# Autodesk Inventor assembly: Funnel Wheel Clamp V4
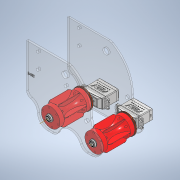
[picture p0: Inventor's stored thumbnail of the model, 180x180]
Saved by Autodesk Inventor 2022 (Build 260153000, 153)
## iProperties
Created: 2022-09-17
Part Number: Funnel Wheel Clamp V4
Document SubType Name: Assembly
Designer: matt
Author: matt
## Documents named in this file (10)
- C:\Users\matt\Documents\Inventor\FTC\2022-23 FTC\Intake\Funnel Wheel Clamp V4.iam
- C:\Users\matt\Documents\Inventor\FTC\2022-23 FTC\FTC Robot Parts\Structural\8mm Bearing with Hex Insert_MIR.iam
- C:\Users\matt\Documents\Inventor\FTC\2022-23 FTC\FTC Robot Parts\Shafts\5mm hex shaft_MIR.ipt
- C:\Users\matt\Documents\Inventor\FTC\2022-23 FTC\FTC Robot Parts\Servos\Servo Horn_MIR.ipt
- C:\Users\matt\Documents\Inventor\FTC\2022-23 FTC\Fasteners\M3 x 8 Button Head.ipt
- C:\Users\matt\Documents\Inventor\FTC\2022-23 FTC\Field\am-4801_Blue Cone.ipt
- C:\Users\matt\Documents\Inventor\FTC\2022-23 FTC\Intake\Intake Sides V5_servo.ipt
- C:\Users\matt\Documents\Inventor\FTC\2022-23 FTC\Motors\REV Smart Servo.ipt
- C:\Users\matt\Documents\Inventor\FTC\2022-23 FTC\Intake\Intake Sides V6ipt.ipt
- C:\Users\matt\Documents\Inventor\FTC\2022-23 FTC\Wheels\Custom Intake Wheel V4.ipt
## Components (19 placed, 9 different names)
1. 8mm Bearing with Hex Insert_MIR:1 [sub-assembly] — Flush:6, Mate:55, Mate:71, Mate:78, Mate:115
2. 8mm Bearing with Hex Insert_MIR:2 [sub-assembly] — Flush:5, Mate:54, Mate:75, Mate:114
3. 5mm hex shaft_MIR:1 — Flush:5, Mate:54, Mate:75, Mate:92
4. 5mm hex shaft_MIR:2 — Flush:6, Mate:55, Mate:71, Mate:72, Mate:93
5. Servo Horn_MIR:1 — Mate:33, Mate:35, Mate:36, Mate:37, Mate:38, Mate:39, Mate:64, Mate:86, Mate:90, Mate:91, Mate:113
6. Servo Horn_MIR:2 — Mate:67, Mate:68, Mate:69, Mate:87, Mate:110
7. M3 x 8 Button Head:1 — Flush:6, Mate:38
8. M3 x 8 Button Head:2 — Flush:6, Flush:7, Mate:39
9. M3 x 8 Button Head:3 — Flush:7, Flush:8, Mate:37
10. M3 x 8 Button Head:4 — Flush:8, Flush:9, Mate:36
11. M3 x 8 Button Head:5 — Flush:9, Flush:10, Mate:35
12. M3 x 8 Button Head:6 — Flush:10, Mate:33, Mate:90
13. Custom Intake Wheel V4:1 — Mate:67, Mate:68, Mate:69, Mate:114
14. Custom Intake Wheel V4:2 — Mate:64, Mate:72, Mate:78, Flush:14, Mate:113
15. am-4801_Blue Cone:1 — Mate:81, Mate:94
16. Intake Sides V5_servo:2 — Mate:88, Mate:89, Mate:95, Mate:96, Mate:107, Mate:108, Flush:15, Flush:16
17. REV Smart Servo:1 — Mate:87, Mate:89, Mate:96, Mate:108, Mate:110
18. REV Smart Servo:2 — Mate:86, Mate:88, Mate:91, Mate:95, Mate:107
19. Intake Sides V6ipt:1 — Mate:115, Flush:15, Flush:16
## Relationships (44: Mate 34, Flush 10)
- Flush:5: 8mm Bearing with Hex Insert_MIR:2 ↔ 5mm hex shaft_MIR:1
- Flush:6: 8mm Bearing with Hex Insert_MIR:1 ↔ 5mm hex shaft_MIR:2
- Flush:6: M3 x 8 Button Head:1 ↔ M3 x 8 Button Head:2
- Flush:7: M3 x 8 Button Head:2 ↔ M3 x 8 Button Head:3
- Flush:8: M3 x 8 Button Head:3 ↔ M3 x 8 Button Head:4
- Flush:9: M3 x 8 Button Head:4 ↔ M3 x 8 Button Head:5
- Flush:10: M3 x 8 Button Head:5 ↔ M3 x 8 Button Head:6
- Mate:33: Servo Horn_MIR:1 ↔ M3 x 8 Button Head:6
- Mate:35: Servo Horn_MIR:1 ↔ M3 x 8 Button Head:5
- Mate:36: Servo Horn_MIR:1 ↔ M3 x 8 Button Head:4
- Mate:37: Servo Horn_MIR:1 ↔ M3 x 8 Button Head:3
- Mate:38: Servo Horn_MIR:1 ↔ M3 x 8 Button Head:1
- Mate:39: Servo Horn_MIR:1 ↔ M3 x 8 Button Head:2
- Mate:54: 8mm Bearing with Hex Insert_MIR:2 ↔ 5mm hex shaft_MIR:1
- Mate:55: 8mm Bearing with Hex Insert_MIR:1 ↔ 5mm hex shaft_MIR:2
- Mate:64: Servo Horn_MIR:1 ↔ Custom Intake Wheel V4:2
- Mate:67: Servo Horn_MIR:2 ↔ Custom Intake Wheel V4:1
- Mate:68: Servo Horn_MIR:2 ↔ Custom Intake Wheel V4:1
- Mate:69: Servo Horn_MIR:2 ↔ Custom Intake Wheel V4:1
- Mate:71: 8mm Bearing with Hex Insert_MIR:1 ↔ 5mm hex shaft_MIR:2
- Mate:72: 5mm hex shaft_MIR:2 ↔ Custom Intake Wheel V4:2
- Mate:75: 8mm Bearing with Hex Insert_MIR:2 ↔ 5mm hex shaft_MIR:1
- Mate:78: 8mm Bearing with Hex Insert_MIR:1 ↔ Custom Intake Wheel V4:2
- Flush:14 (-32 mm): Custom Intake Wheel V4:2
- Mate:81: am-4801_Blue Cone:1
- Mate:86: Servo Horn_MIR:1 ↔ REV Smart Servo:2
- Mate:87: Servo Horn_MIR:2 ↔ REV Smart Servo:1
- Mate:88: Intake Sides V5_servo:2 ↔ REV Smart Servo:2
- Mate:89: Intake Sides V5_servo:2 ↔ REV Smart Servo:1
- Mate:90: Servo Horn_MIR:1 ↔ M3 x 8 Button Head:6
- Mate:91: Servo Horn_MIR:1 ↔ REV Smart Servo:2
- Mate:92: 5mm hex shaft_MIR:1
- Mate:93: 5mm hex shaft_MIR:2
- Mate:94: am-4801_Blue Cone:1
- Mate:95: Intake Sides V5_servo:2 ↔ REV Smart Servo:2
- Mate:96: Intake Sides V5_servo:2 ↔ REV Smart Servo:1
- Mate:107: Intake Sides V5_servo:2 ↔ REV Smart Servo:2
- Mate:108: Intake Sides V5_servo:2 ↔ REV Smart Servo:1
- Mate:110: Servo Horn_MIR:2 ↔ REV Smart Servo:1
- Mate:113: Servo Horn_MIR:1 ↔ Custom Intake Wheel V4:2
- Mate:114: 8mm Bearing with Hex Insert_MIR:2 ↔ Custom Intake Wheel V4:1
- Mate:115: 8mm Bearing with Hex Insert_MIR:1 ↔ Intake Sides V6ipt:1
- Flush:15: Intake Sides V5_servo:2 ↔ Intake Sides V6ipt:1
- Flush:16: Intake Sides V5_servo:2 ↔ Intake Sides V6ipt:1
